# Autodesk Inventor assembly: Caja
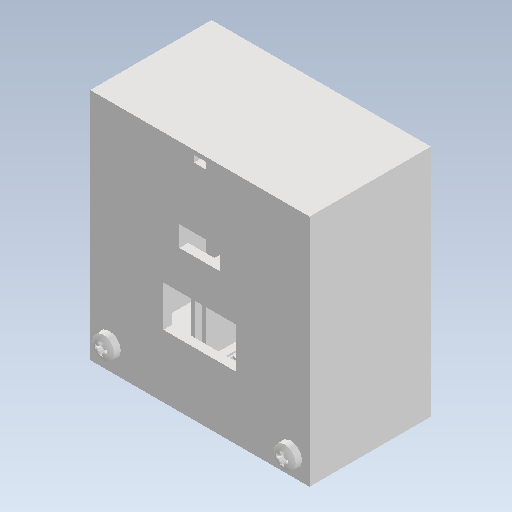
[picture p0: Inventor's stored thumbnail of the model, 512x512]
Saved by Autodesk Inventor 2021 (Build 250183000, 183)
## iProperties
Created: 2023-09-03
Part Number: Caja
Document SubType Name: Assembly
Designer: Sergio
Author: Sergio
## Documents named in this file (4)
- D:\Sergio\OneDrive - Escuela Superior Politécnica del Litoral\Documentos\12vo Semestre (último)\Diseño Mecatrónico\Proyecto\Diseño Mecánico\solucion GANADORA\Caja\Caja.iam
- D:\Sergio\OneDrive - Escuela Superior Politécnica del Litoral\Documentos\12vo Semestre (último)\Diseño Mecatrónico\Proyecto\Diseño Mecánico\solucion GANADORA\Caja\Cuerpo de caja.ipt
- D:\Sergio\OneDrive - Escuela Superior Politécnica del Litoral\Documentos\12vo Semestre (último)\Diseño Mecatrónico\Proyecto\Diseño Mecánico\solucion GANADORA\Caja\Tapa de caja.ipt
- D:\Sergio\Documents\Inventor\Content Center Files\R2021\es-ES\DIN 7985 (H)\DIN 7985 (H) - M4x10-H.ipt
## Components (4 placed, 3 different names)
1. Cuerpo de caja:1 — Coincidencia:1, Coincidencia:2, Coincidencia:3
2. Tapa de caja:1 — Coincidencia:1, Coincidencia:2, Coincidencia:3, Coincidencia:4, Coincidencia:5, Coincidencia:6, Coincidencia:7
3. DIN 7985 (H) M4x10-H:1 — Coincidencia:4, Coincidencia:5
4. DIN 7985 (H) M4x10-H:2 — Coincidencia:6, Coincidencia:7
## Relationships (7: Mate 7)
- Coincidencia:1 [Mate]: Cuerpo de caja:1 ↔ Tapa de caja:1
- Coincidencia:2 [Mate]: Cuerpo de caja:1 ↔ Tapa de caja:1
- Coincidencia:3 [Mate]: Cuerpo de caja:1 ↔ Tapa de caja:1
- Coincidencia:4 [Mate]: Tapa de caja:1 ↔ DIN 7985 (H) M4x10-H:1
- Coincidencia:5 [Mate]: Tapa de caja:1 ↔ DIN 7985 (H) M4x10-H:1
- Coincidencia:6 [Mate]: Tapa de caja:1 ↔ DIN 7985 (H) M4x10-H:2
- Coincidencia:7 [Mate]: Tapa de caja:1 ↔ DIN 7985 (H) M4x10-H:2
